# Autodesk Inventor assembly: Side Panel
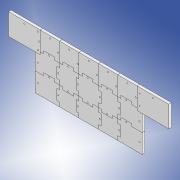
[picture p0: Inventor's stored thumbnail of the model, 180x180]
Saved by Autodesk Inventor 2017 SP1 (Build 210196100, 196)
## iProperties
Created: 2017-08-09
Part Number: Side Panel
Document SubType Name: Assembly
Designer: Zach
Author: Zach
## Documents named in this file (14)
- C:\Users\Zach\Documents\GitHub\cr-laundry-robot\src\Base\Side Panel\Side Panel Front.iam
- C:\Users\Zach\Documents\GitHub\cr-laundry-robot\src\Base\Side Panel\SP001.ipt
- C:\Users\Zach\Documents\GitHub\cr-laundry-robot\src\Base\Side Panel\SP002.ipt
- C:\Users\Zach\Documents\GitHub\cr-laundry-robot\src\Base\Side Panel\SP003.ipt
- C:\Users\Zach\Documents\GitHub\cr-laundry-robot\src\Base\Side Panel\SP004.ipt
- C:\Users\Zach\Documents\GitHub\cr-laundry-robot\src\Base\Side Panel\SP005.ipt
- C:\Users\Zach\Documents\GitHub\cr-laundry-robot\src\Base\Side Panel\SP007.ipt
- C:\Users\Zach\Documents\GitHub\cr-laundry-robot\src\Base\Side Panel\SP006.ipt
- C:\Users\Zach\Documents\GitHub\cr-laundry-robot\src\Base\Side Panel\SP008.ipt
- C:\Users\Zach\Documents\GitHub\cr-laundry-robot\src\Base\Side Panel\SP009.ipt
- C:\Users\Zach\Documents\GitHub\cr-laundry-robot\src\Base\Side Panel\SP010.ipt
- C:\Users\Zach\Documents\GitHub\cr-laundry-robot\src\Base\Side Panel\SP011.ipt
- C:\Users\Zach\Documents\GitHub\cr-laundry-robot\src\Base\Side Panel\SP012.ipt
- C:\Users\Zach\Documents\GitHub\cr-laundry-robot\src\Base\Side Panel\SP013.ipt
## Components (17 placed, 13 different names)
1. SP001:1 — Mate:1, Mate:2
2. SP002:1 — Mate:1, Mate:2, Mate:3, Mate:4, Mate:5, Mate:6
3. SP003:1 — Mate:3, Mate:4, Mate:17, Mate:18, Mate:31
4. SP002:2 — Mate:5, Mate:6, Mate:7, Mate:8
5. SP002:3 — Mate:7, Mate:8, Mate:9, Mate:10, Mate:36
6. SP002:4 — Mate:9, Mate:10, Mate:11, Mate:12, Mate:34
7. SP002:5 — Mate:11, Mate:12, Mate:13, Mate:14, Mate:15, Mate:16
8. SP004:1 — Mate:13, Mate:14
9. SP005:1 — Mate:15, Mate:16, Mate:19, Mate:20
10. SP006:1 — Mate:17, Mate:18, Mate:21, Mate:22
11. SP007:1 — Mate:19, Mate:20, Mate:23, Mate:24
12. SP008:1 — Mate:21, Mate:22, Mate:26, Mate:33
13. SP009:1 — Mate:23, Mate:24, Mate:25, Mate:27, Mate:35
14. SP010:1 — Mate:25, Mate:26, Mate:27, Mate:37, Mate:38
15. SP011:2 — Mate:31, Mate:33
16. SP012:1 — Mate:34, Mate:35
17. SP013:1 — Mate:36, Mate:37, Mate:38
## Relationships (34: Mate 34)
- Mate:1: SP001:1 ↔ SP002:1
- Mate:2: SP001:1 ↔ SP002:1
- Mate:3: SP002:1 ↔ SP003:1
- Mate:4: SP002:1 ↔ SP003:1
- Mate:5: SP002:1 ↔ SP002:2
- Mate:6: SP002:1 ↔ SP002:2
- Mate:7: SP002:2 ↔ SP002:3
- Mate:8: SP002:2 ↔ SP002:3
- Mate:9: SP002:3 ↔ SP002:4
- Mate:10: SP002:3 ↔ SP002:4
- Mate:11: SP002:4 ↔ SP002:5
- Mate:12: SP002:4 ↔ SP002:5
- Mate:13: SP002:5 ↔ SP004:1
- Mate:14: SP002:5 ↔ SP004:1
- Mate:15: SP002:5 ↔ SP005:1
- Mate:16: SP002:5 ↔ SP005:1
- Mate:17: SP003:1 ↔ SP006:1
- Mate:18: SP003:1 ↔ SP006:1
- Mate:19: SP005:1 ↔ SP007:1
- Mate:20: SP005:1 ↔ SP007:1
- Mate:21: SP006:1 ↔ SP008:1
- Mate:22: SP006:1 ↔ SP008:1
- Mate:23: SP007:1 ↔ SP009:1
- Mate:24: SP007:1 ↔ SP009:1
- Mate:25: SP009:1 ↔ SP010:1
- Mate:26: SP008:1 ↔ SP010:1
- Mate:27: SP009:1 ↔ SP010:1
- Mate:31: SP003:1 ↔ SP011:2
- Mate:33: SP008:1 ↔ SP011:2
- Mate:34: SP002:4 ↔ SP012:1
- Mate:35: SP009:1 ↔ SP012:1
- Mate:36: SP002:3 ↔ SP013:1
- Mate:37: SP010:1 ↔ SP013:1
- Mate:38: SP010:1 ↔ SP013:1
